# Autodesk Inventor assembly: ASY NVPH-600 reagent tank
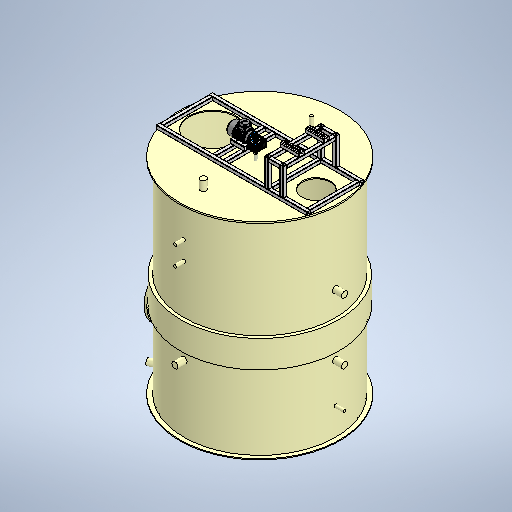
[picture p0: Inventor's stored thumbnail of the model, 512x512]
Saved by Autodesk Inventor 2025.1 (Build 291241020, 241B)
## iProperties
Created: 2025-04-01
Part Number: ASY NVPH-600 reagent tank
Document SubType Name: Assembly
Designer: user
Author: user
## Documents named in this file (5)
- C:\Users\user\YandexDisk-badmisterfox\home pc\Inventor\NDM-VOS_powder_hopper\ASY NVPH-600 reagent tank.iam
- C:\Users\user\YandexDisk-badmisterfox\home pc\Inventor\NDM-VOS_powder_hopper\NDM-VOS dummy3.ipt
- C:\Users\user\YandexDisk-badmisterfox\home pc\Inventor\NDM-VOS_powder_hopper\3d party\motor-reductor NMRV040\motor-reductor NMRV040.iam
- C:\Users\user\YandexDisk-badmisterfox\home pc\Inventor\NDM-VOS_powder_hopper\3d party\Mixer 22.04.24\ASY mixer 3.iam
- C:\Users\user\YandexDisk-badmisterfox\home pc\Inventor\NDM-VOS_powder_hopper\ASY HPR 290 Support Frame.iam
## Components (4 placed, 4 different names)
1. NDM-VOS dummy3:1
2. motor-reductor NMRV040:1 [sub-assembly]
3. ASY mixer 3:1 [sub-assembly]
4. ASY HPR 290 Support Frame:1 [sub-assembly]
## Relationships (5: Flush 2, Mate 1, RevoluteJoint 1, WeldJoint 1)
- [Flush]: NDM-VOS dummy3:1 ↔ ASY HPR 290 Support Frame:1
- [Mate]: NDM-VOS dummy3:1 ↔ ASY HPR 290 Support Frame:1
- [Flush]: NDM-VOS dummy3:1 ↔ ASY HPR 290 Support Frame:1
- [RevoluteJoint]: motor-reductor NMRV040:1 ↔ ASY mixer 3:1
- [WeldJoint]: motor-reductor NMRV040:1 ↔ ASY HPR 290 Support Frame:1
